# Autodesk Inventor assembly: tEST
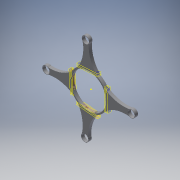
[picture p0: Inventor's stored thumbnail of the model, 180x180]
Saved by Autodesk Inventor 2017 (Build 210142000, 142)
## iProperties
Part Number: tEST
Material: Générique
Document SubType Name: Assembly
Designer: Thomas
Author: Thomas
## Documents named in this file (3)
- C:\Users\Thomas\Documents\Modele 3D\Drone\tEST.iam
- C:\Users\Thomas\Documents\Modele 3D\Drone\Aile.ipt
- C:\Users\Thomas\Documents\Modele 3D\Drone\Attache centre.ipt
## Components (5 placed, 2 different names)
1. Aile:1 — Affleurement:1, Placage:1, Affleurement:4
2. Attache centre:1 — Affleurement:1, Placage:1, Placage:2, Placage:3, Placage:4, Affleurement:2, Affleurement:3, Affleurement:4, Affleurement:5, Placage:5
3. Aile:2 — Placage:2, Affleurement:3
4. Aile:3 — Placage:4, Affleurement:5
5. Aile:4 — Placage:3, Affleurement:2, Placage:5
## Relationships (10: Flush 5, Mate 5)
- Affleurement:1 [Flush]: Aile:1 ↔ Attache centre:1
- Placage:1 [Mate]: Aile:1 ↔ Attache centre:1
- Placage:2 [Mate]: Attache centre:1 ↔ Aile:2
- Placage:3 [Mate]: Attache centre:1 ↔ Aile:4
- Placage:4 [Mate]: Attache centre:1 ↔ Aile:3
- Affleurement:2 [Flush]: Attache centre:1 ↔ Aile:4
- Affleurement:3 [Flush]: Attache centre:1 ↔ Aile:2
- Affleurement:4 [Flush]: Aile:1 ↔ Attache centre:1
- Affleurement:5 [Flush]: Attache centre:1 ↔ Aile:3
- Placage:5 [Mate]: Attache centre:1 ↔ Aile:4
